# Autodesk Inventor assembly: 01 ASY GBK wall shield 1.1.1
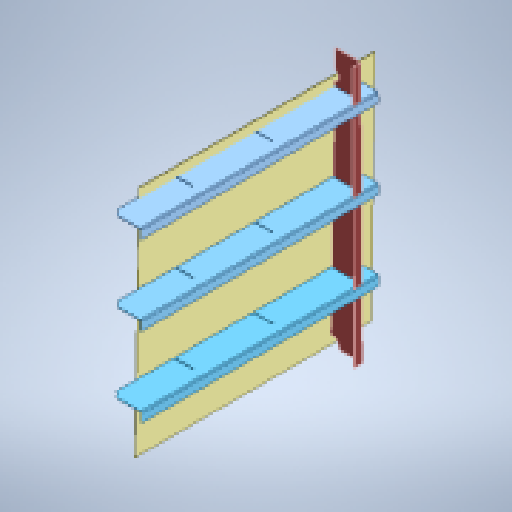
[picture p0: Inventor's stored thumbnail of the model, 512x512]
Saved by Autodesk Inventor 2026 (Build 300175000, 175)
## iProperties
Created: 2026-05-07
Part Number: 01 ASY GBK wall shield 1.1.1
Document SubType Name: Assembly
Designer: admin
Mass: 245734 g
Surface Area: 167509 cm^2
Volume: 31303.7 cm^3
Density: 7.85 g/cm^3
Author: admin
## Documents named in this file (6)
- C:\Users\pokla\Documents\Inventor\GBK-Gubkinskiy\01 ASY GBK wall shield 1.1.1.iam
- C:\Users\pokla\Documents\Inventor\GBK-Gubkinskiy\01.1 GBK shield.ipt
- C:\Users\pokla\Documents\Inventor\GBK-Gubkinskiy\01.2 GBK main rib.ipt
- C:\Users\pokla\Documents\Inventor\GBK-Gubkinskiy\01.3 GBK stringer 1.ipt
- C:\Users\pokla\Documents\Inventor\GBK-Gubkinskiy\0232 GBK stringer 2.ipt
- C:\Users\pokla\Documents\Inventor\GBK-Gubkinskiy\0233 GBK stringer 3.ipt
## Components (7 placed, 6 different names)
1. 0232 GBK stringer 2:1
2. 0233 GBK stringer 3:1
3. 01.3 GBK stringer 1.ipt:1
4. 01.1 GBK shield.ipt:1
5. 01.2 GBK main rib.ipt:1
6. 01.2 GBK main rib:2
7. 01.2 GBK main rib:3
## Component patterns: (3 elements, first: 01.2 GBK main rib.ipt:1)
## Relationships (6: WeldJoint 3, Mate 2, Flush 1)
- [Mate]: 01.1 GBK shield.ipt:1 ↔ 01.2 GBK main rib.ipt:1
- [Flush] (250 mm): 01.1 GBK shield.ipt:1 ↔ 01.2 GBK main rib.ipt:1
- [Mate]: 01.1 GBK shield.ipt:1 ↔ 01.2 GBK main rib.ipt:1
- [WeldJoint] (4 mm): 01.3 GBK stringer 1.ipt:1 ↔ 01.2 GBK main rib.ipt:1
- [WeldJoint] (4 mm): 0232 GBK stringer 2:1 ↔ 01.2 GBK main rib.ipt:1
- [WeldJoint] (4 mm): 0233 GBK stringer 3:1 ↔ 01.2 GBK main rib.ipt:1
